(part 1 of 2)
# Autodesk Inventor assembly: Functioning Test Chasis
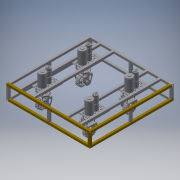
[picture p0: Inventor's stored thumbnail of the model, 180x180]
Saved by Autodesk Inventor 2019 (Build 230136000, 136)
## iProperties
has-driver: False
num-sensors: 0
has-driver: True
driver-type: 1
motor-type: 0
driver-port1: 1
driver-port2: -1
driver-isCan: False
driver-lowerLimit: 0.0
driver-upperLimit: 0.0
driver-inputGear: 0.0
driver-outputGear: 0.0
driver-hasBrake: False
has-wheel: True
wheel-type: 3
wheel-isDriveWheel: True
wheel-frictionLevel: 1
has-pneumatic: False
has-elevator: False
driver-port1: 0
Created: 2019-01-14
Part Number: Functioning Test Chasis
Document SubType Name: Assembly
Designer: josh
robot-name: Chasis
robot-weight-kg: 222.26052856445312
robot-prefer-metric: False
robot-driveTrainType: 1
Author: josh
## Documents named in this file (36)
- D:\Synthesis Robots\Epsilon\Functioning Test Chasis.iam
- D:\Synthesis Robots\Epsilon\Chasis.iam
- D:\Synthesis Robots\Epsilon\4 in HiGrip Wheel.iam
- D:\Synthesis Robots\Epsilon\FR6ZZ-L Hex Bearing.ipt
- D:\Synthesis Robots\Epsilon\375 Hex Output Shaft Rev 2.ipt
- D:\Synthesis Robots\Epsilon\375 Hex Hub.ipt
- D:\Synthesis Robots\Epsilon\10-24 Hex Washer Rolling x 3-4_93882A213.ipt
- D:\Synthesis Robots\Epsilon\125x443 spacer SPS-0750-0443-0125.ipt
- D:\Synthesis Robots\Epsilon\375 E-klip - Mcm 97431A320_97431A320.ipt
- D:\Synthesis Robots\Epsilon\20t 1-25mod bevel gear.ipt
- D:\Synthesis Robots\Epsilon\40t 1-25mod bevel gear.ipt
- D:\Synthesis Robots\Epsilon\AMS C Housing Rev 2.ipt
- D:\Synthesis Robots\Epsilon\10-32 Nylock Nut 1_90631A411.ipt
- D:\Synthesis Robots\Epsilon\10-32x1250_shcs.ipt
- D:\Synthesis Robots\Epsilon\620x215 alum spacer 83062 K-S.ipt
- D:\Synthesis Robots\Epsilon\Bevel Input Shaft.ipt
- D:\Synthesis Robots\Epsilon\FR8ZZ Bearing_smart.ipt
- D:\Synthesis Robots\Epsilon\FR6ZZ Bearing_smart.ipt
- D:\Synthesis Robots\Epsilon\12T CIM Shaft.ipt
- D:\Synthesis Robots\Epsilon\Gear Plate.ipt
- D:\Synthesis Robots\Epsilon\40T 20dp 375h_Inch - Spur gear 20DP 40T 14.5PA .372FW ---S40N3.0H2.0L0.25N.ipt
- D:\Synthesis Robots\Epsilon\500 Washer am-1001.ipt
- D:\Synthesis Robots\Epsilon\10-32x0625_shcs_HX-SHCS 0.19-32x1.375x1-C.ipt
- D:\Synthesis Robots\Epsilon\1100x215 alum spacer 83062 K-S.ipt
- D:\Synthesis Robots\Epsilon\10-32 Nylock Nut.ipt
- D:\Synthesis Robots\Epsilon\10-32x1750_shcs_HX-SHCS 0.19-32x1.375x1-C.ipt
- D:\Synthesis Robots\Epsilon\Bearing Plate.ipt
- D:\Synthesis Robots\Epsilon\40T Sleeve Gear REV2.ipt
- D:\Synthesis Robots\Epsilon\VEX 217-2736 0500 Collar Clamp.ipt
- D:\Synthesis Robots\Epsilon\CIM Motor SW.ipt
- D:\Synthesis Robots\Epsilon\Motor Mount Plate Rev 2.ipt
- D:\Synthesis Robots\Epsilon\48T 10mm bore gear.ipt
- D:\Synthesis Robots\Epsilon\PG-71.ipt
- D:\Synthesis Robots\Epsilon\SHCS M4x10_91290A187.ipt
- D:\Synthesis Robots\Epsilon\438x406 spacer 13RS100043.ipt
- D:\Synthesis Robots\Epsilon\375 External Self Locking Ring_98430A134.ipt
## Components (273 placed, 35 different names)
1. Chasis:1 [sub-assembly] — Mate:253, Flush:23, Mate:254, Mate:505, Flush:46, Mate:506, Mate:507, Flush:47, Mate:508, Mate:634, Flush:59, Mate:635
2. 4 in HiGrip Wheel:2 [sub-assembly]
3. Bevel Input Shaft:2
4. AMS C Housing Rev 2:2
5. FR6ZZ-L Hex Bearing:4
6. 20t 1-25mod bevel gear:2
7. 375 Hex Output Shaft Rev 2:2
8. 375 Hex Hub:2
9. 10-24 Hex Washer Rolling x 3-4_93882A213:7
10. 10-24 Hex Washer Rolling x 3-4_93882A213:8
11. 10-24 Hex Washer Rolling x 3-4_93882A213:9
12. 10-24 Hex Washer Rolling x 3-4_93882A213:10
13. 10-24 Hex Washer Rolling x 3-4_93882A213:11
14. 10-24 Hex Washer Rolling x 3-4_93882A213:12
15. 125x443 spacer SPS-0750-0443-0125:2
16. 375 E-klip - Mcm 97431A320_97431A320:2
17. 40t 1-25mod bevel gear:2
18. FR8ZZ Bearing_smart:2
19. 12T CIM Shaft:2
20. 10-32 Nylock Nut 1_90631A411:5
21. 10-32 Nylock Nut 1_90631A411:6
22. 10-32 Nylock Nut 1_90631A411:7
23. 10-32 Nylock Nut 1_90631A411:8
24. 10-32x1250_shcs:5
25. 10-32x1250_shcs:6
26. 10-32x1250_shcs:7
27. 10-32x1250_shcs:8
28. 620x215 alum spacer 83062 K-S:5
29. 620x215 alum spacer 83062 K-S:6
30. 620x215 alum spacer 83062 K-S:7
31. 620x215 alum spacer 83062 K-S:8
32. FR6ZZ Bearing_smart:3
33. Gear Plate:2
34. 40T 20dp 375h_Inch - Spur gear 20DP 40T 14.5PA .372FW ---S40N3.0H2.0L0.25N:2
35. 500 Washer am-1001:3
36. 500 Washer am-1001:4
37. FR6ZZ Bearing_smart:4
38. 10-32x0625_shcs_HX-SHCS 0.19-32x1.375x1-C:7
39. 10-32x0625_shcs_HX-SHCS 0.19-32x1.375x1-C:8
40. 10-32x0625_shcs_HX-SHCS 0.19-32x1.375x1-C:9
41. 10-32x0625_shcs_HX-SHCS 0.19-32x1.375x1-C:10
42. 40T Sleeve Gear REV2:2
43. PG-71:2
44. 48T 10mm bore gear:2
45. 375 External Self Locking Ring_98430A134:2
46. 438x406 spacer 13RS100043:2
47. SHCS M4x10_91290A187:8
48. SHCS M4x10_91290A187:7
49. SHCS M4x10_91290A187:6
50. SHCS M4x10_91290A187:5
51. 10-32x0625_shcs_HX-SHCS 0.19-32x1.375x1-C:12
52. 10-32x0625_shcs_HX-SHCS 0.19-32x1.375x1-C:11
53. Motor Mount Plate Rev 2:2 — Mate:253, Flush:23, Mate:254
54. CIM Motor SW:2
55. VEX 217-2736 0500 Collar Clamp:2
56. Bearing Plate:2
57. 10-32 Nylock Nut:8
58. 10-32 Nylock Nut:7
59. 10-32 Nylock Nut:6
60. 10-32x1750_shcs_HX-SHCS 0.19-32x1.375x1-C:8
61. 10-32x1750_shcs_HX-SHCS 0.19-32x1.375x1-C:7
62. 10-32x1750_shcs_HX-SHCS 0.19-32x1.375x1-C:6
63. 1100x215 alum spacer 83062 K-S:8
64. 1100x215 alum spacer 83062 K-S:7
65. 1100x215 alum spacer 83062 K-S:6
66. 10-32x1750_shcs_HX-SHCS 0.19-32x1.375x1-C:5
67. 10-32 Nylock Nut:5
68. 1100x215 alum spacer 83062 K-S:5
69. FR6ZZ-L Hex Bearing:3
70. FR6ZZ-L Hex Bearing:5
71. FR6ZZ-L Hex Bearing:6
72. 375 Hex Output Shaft Rev 2:3
73. 375 Hex Hub:3
74. 10-24 Hex Washer Rolling x 3-4_93882A213:13
75. 10-24 Hex Washer Rolling x 3-4_93882A213:14
76. 10-24 Hex Washer Rolling x 3-4_93882A213:15
77. 10-24 Hex Washer Rolling x 3-4_93882A213:16
78. 10-24 Hex Washer Rolling x 3-4_93882A213:17
79. 10-24 Hex Washer Rolling x 3-4_93882A213:18
80. 125x443 spacer SPS-0750-0443-0125:3
81. 375 E-klip - Mcm 97431A320_97431A320:3
82. 20t 1-25mod bevel gear:3
83. 40t 1-25mod bevel gear:3
84. AMS C Housing Rev 2:3
85. 10-32 Nylock Nut 1_90631A411:9
86. 10-32 Nylock Nut 1_90631A411:10
87. 10-32 Nylock Nut 1_90631A411:11
88. 10-32 Nylock Nut 1_90631A411:12
89. 10-32x1250_shcs:9
90. 10-32x1250_shcs:10
91. 10-32x1250_shcs:11
92. 10-32x1250_shcs:12
93. 620x215 alum spacer 83062 K-S:9
94. 620x215 alum spacer 83062 K-S:10
95. 620x215 alum spacer 83062 K-S:11
96. 620x215 alum spacer 83062 K-S:12
97. Bevel Input Shaft:3
98. FR8ZZ Bearing_smart:3
99. FR6ZZ Bearing_smart:5
100. 12T CIM Shaft:3
101. Gear Plate:3
102. 40T 20dp 375h_Inch - Spur gear 20DP 40T 14.5PA .372FW ---S40N3.0H2.0L0.25N:3
103. 500 Washer am-1001:5
104. 500 Washer am-1001:6
105. FR6ZZ Bearing_smart:6
106. 10-32x0625_shcs_HX-SHCS 0.19-32x1.375x1-C:13
107. 10-32x0625_shcs_HX-SHCS 0.19-32x1.375x1-C:14
108. 10-32x0625_shcs_HX-SHCS 0.19-32x1.375x1-C:15
109. 10-32x0625_shcs_HX-SHCS 0.19-32x1.375x1-C:16
110. 1100x215 alum spacer 83062 K-S:9
111. 10-32 Nylock Nut:9
112. 10-32x1750_shcs_HX-SHCS 0.19-32x1.375x1-C:9
113. 1100x215 alum spacer 83062 K-S:10
114. 1100x215 alum spacer 83062 K-S:11
115. 1100x215 alum spacer 83062 K-S:12
116. 10-32x1750_shcs_HX-SHCS 0.19-32x1.375x1-C:10
117. 10-32x1750_shcs_HX-SHCS 0.19-32x1.375x1-C:11
118. 10-32x1750_shcs_HX-SHCS 0.19-32x1.375x1-C:12
119. 10-32 Nylock Nut:10
120. 10-32 Nylock Nut:11
121. 10-32 Nylock Nut:12
122. Bearing Plate:3
123. 40T Sleeve Gear REV2:3
124. VEX 217-2736 0500 Collar Clamp:3
125. CIM Motor SW:3
126. Motor Mount Plate Rev 2:3 — Mate:505, Flush:46, Mate:506
127. 48T 10mm bore gear:3
128. 10-32x0625_shcs_HX-SHCS 0.19-32x1.375x1-C:17
129. 10-32x0625_shcs_HX-SHCS 0.19-32x1.375x1-C:18
130. PG-71:3
131. SHCS M4x10_91290A187:9
132. SHCS M4x10_91290A187:10
133. SHCS M4x10_91290A187:11
134. SHCS M4x10_91290A187:12
135. 438x406 spacer 13RS100043:3
136. 375 External Self Locking Ring_98430A134:3
137. 4 in HiGrip Wheel:3 [sub-assembly]
138. FR6ZZ-L Hex Bearing:7
139. FR6ZZ-L Hex Bearing:8
140. 375 Hex Output Shaft Rev 2:4
141. 375 Hex Hub:4
142. 10-24 Hex Washer Rolling x 3-4_93882A213:19
143. 10-24 Hex Washer Rolling x 3-4_93882A213:20
144. 10-24 Hex Washer Rolling x 3-4_93882A213:21
145. 10-24 Hex Washer Rolling x 3-4_93882A213:22
146. 10-24 Hex Washer Rolling x 3-4_93882A213:23
147. 10-24 Hex Washer Rolling x 3-4_93882A213:24
148. 125x443 spacer SPS-0750-0443-0125:4
149. 375 E-klip - Mcm 97431A320_97431A320:4
150. 20t 1-25mod bevel gear:4
151. 40t 1-25mod bevel gear:4
152. AMS C Housing Rev 2:4
153. 10-32 Nylock Nut 1_90631A411:13
154. 10-32 Nylock Nut 1_90631A411:14
155. 10-32 Nylock Nut 1_90631A411:15
156. 10-32 Nylock Nut 1_90631A411:16
157. 10-32x1250_shcs:13
158. 10-32x1250_shcs:14
159. 10-32x1250_shcs:15
160. 10-32x1250_shcs:16
161. 620x215 alum spacer 83062 K-S:13
162. 620x215 alum spacer 83062 K-S:14
163. 620x215 alum spacer 83062 K-S:15
164. 620x215 alum spacer 83062 K-S:16
165. Bevel Input Shaft:4
166. FR8ZZ Bearing_smart:4
167. FR6ZZ Bearing_smart:7
168. 12T CIM Shaft:4
169. Gear Plate:4
170. 40T 20dp 375h_Inch - Spur gear 20DP 40T 14.5PA .372FW ---S40N3.0H2.0L0.25N:4
171. 500 Washer am-1001:7
172. 500 Washer am-1001:8
173. FR6ZZ Bearing_smart:8
174. 10-32x0625_shcs_HX-SHCS 0.19-32x1.375x1-C:19
175. 10-32x0625_shcs_HX-SHCS 0.19-32x1.375x1-C:20
176. 10-32x0625_shcs_HX-SHCS 0.19-32x1.375x1-C:21
177. 10-32x0625_shcs_HX-SHCS 0.19-32x1.375x1-C:22
178. 1100x215 alum spacer 83062 K-S:13
179. 10-32 Nylock Nut:13
180. 10-32x1750_shcs_HX-SHCS 0.19-32x1.375x1-C:13
181. 1100x215 alum spacer 83062 K-S:14
182. 1100x215 alum spacer 83062 K-S:15
183. 1100x215 alum spacer 83062 K-S:16
184. 10-32x1750_shcs_HX-SHCS 0.19-32x1.375x1-C:14
185. 10-32x1750_shcs_HX-SHCS 0.19-32x1.375x1-C:15
186. 10-32x1750_shcs_HX-SHCS 0.19-32x1.375x1-C:16
187. 10-32 Nylock Nut:14
188. 10-32 Nylock Nut:15
189. 10-32 Nylock Nut:16
190. Bearing Plate:4
191. 40T Sleeve Gear REV2:4
192. VEX 217-2736 0500 Collar Clamp:4
193. CIM Motor SW:4
194. Motor Mount Plate Rev 2:4 — Mate:507, Flush:47, Mate:508
195. 48T 10mm bore gear:4
196. 10-32x0625_shcs_HX-SHCS 0.19-32x1.375x1-C:23
197. 10-32x0625_shcs_HX-SHCS 0.19-32x1.375x1-C:24
198. PG-71:4
199. SHCS M4x10_91290A187:13
200. SHCS M4x10_91290A187:14
201. SHCS M4x10_91290A187:15
202. SHCS M4x10_91290A187:16
203. 438x406 spacer 13RS100043:4
204. 375 External Self Locking Ring_98430A134:4
205. 4 in HiGrip Wheel:4 [sub-assembly]
206. FR6ZZ-L Hex Bearing:9
207. FR6ZZ-L Hex Bearing:10
208. 375 Hex Output Shaft Rev 2:5
209. 375 Hex Hub:5
210. 10-24 Hex Washer Rolling x 3-4_93882A213:25
211. 10-24 Hex Washer Rolling x 3-4_93882A213:26
212. 10-24 Hex Washer Rolling x 3-4_93882A213:27
213. 10-24 Hex Washer Rolling x 3-4_93882A213:28
214. 10-24 Hex Washer Rolling x 3-4_93882A213:29
215. 10-24 Hex Washer Rolling x 3-4_93882A213:30
216. 125x443 spacer SPS-0750-0443-0125:5
217. 375 E-klip - Mcm 97431A320_97431A320:5
218. 20t 1-25mod bevel gear:5
219. 40t 1-25mod bevel gear:5
220. AMS C Housing Rev 2:5
221. 10-32 Nylock Nut 1_90631A411:17
222. 10-32 Nylock Nut 1_90631A411:18
223. 10-32 Nylock Nut 1_90631A411:19
224. 10-32 Nylock Nut 1_90631A411:20
225. 10-32x1250_shcs:17
226. 10-32x1250_shcs:18
227. 10-32x1250_shcs:19
228. 10-32x1250_shcs:20
229. 620x215 alum spacer 83062 K-S:17
230. 620x215 alum spacer 83062 K-S:18
231. 620x215 alum spacer 83062 K-S:19
232. 620x215 alum spacer 83062 K-S:20
233. Bevel Input Shaft:5
234. FR8ZZ Bearing_smart:5
235. FR6ZZ Bearing_smart:9
236. 12T CIM Shaft:5
237. Gear Plate:5
238. 40T 20dp 375h_Inch - Spur gear 20DP 40T 14.5PA .372FW ---S40N3.0H2.0L0.25N:5
239. 500 Washer am-1001:9
240. 500 Washer am-1001:10
241. FR6ZZ Bearing_smart:10
242. 10-32x0625_shcs_HX-SHCS 0.19-32x1.375x1-C:25
243. 10-32x0625_shcs_HX-SHCS 0.19-32x1.375x1-C:26
244. 10-32x0625_shcs_HX-SHCS 0.19-32x1.375x1-C:27
245. 10-32x0625_shcs_HX-SHCS 0.19-32x1.375x1-C:28
246. 1100x215 alum spacer 83062 K-S:17
247. 10-32 Nylock Nut:17
248. 10-32x1750_shcs_HX-SHCS 0.19-32x1.375x1-C:17
249. 1100x215 alum spacer 83062 K-S:18
250. 1100x215 alum spacer 83062 K-S:19
251. 1100x215 alum spacer 83062 K-S:20
252. 10-32x1750_shcs_HX-SHCS 0.19-32x1.375x1-C:18
253. 10-32x1750_shcs_HX-SHCS 0.19-32x1.375x1-C:19
254. 10-32x1750_shcs_HX-SHCS 0.19-32x1.375x1-C:20
255. 10-32 Nylock Nut:18
256. 10-32 Nylock Nut:19
257. 10-32 Nylock Nut:20
258. Bearing Plate:5
259. 40T Sleeve Gear REV2:5
260. VEX 217-2736 0500 Collar Clamp:5
261. CIM Motor SW:5
262. Motor Mount Plate Rev 2:5 — Mate:634, Flush:59, Mate:635
263. 48T 10mm bore gear:5
264. 10-32x0625_shcs_HX-SHCS 0.19-32x1.375x1-C:29
265. 10-32x0625_shcs_HX-SHCS 0.19-32x1.375x1-C:30
266. PG-71:5
267. SHCS M4x10_91290A187:17
268. SHCS M4x10_91290A187:18
269. SHCS M4x10_91290A187:19
270. SHCS M4x10_91290A187:20
271. 438x406 spacer 13RS100043:5
272. 375 External Self Locking Ring_98430A134:5
273. 4 in HiGrip Wheel:5 [sub-assembly]
## Relationships (592: Mate 508, Flush 48, RevoluteJoint 28, RelateRotation 8)
- [Mate]: 375 Hex Hub:2 ↔ 10-24 Hex Washer Rolling x 3-4_93882A213:12
- [Mate]: 375 Hex Hub:2 ↔ 10-24 Hex Washer Rolling x 3-4_93882A213:7
- [Mate]: 375 Hex Hub:2 ↔ 10-24 Hex Washer Rolling x 3-4_93882A213:11
- [Mate]: 375 Hex Hub:2 ↔ 10-24 Hex Washer Rolling x 3-4_93882A213:10
- [Mate]: 375 Hex Hub:2 ↔ 10-24 Hex Washer Rolling x 3-4_93882A213:9
- [Mate]: 375 Hex Hub:2 ↔ 10-24 Hex Washer Rolling x 3-4_93882A213:8
- [Mate]: 375 Hex Hub:2 ↔ 10-24 Hex Washer Rolling x 3-4_93882A213:8
- [Mate]: 375 Hex Hub:2 ↔ 10-24 Hex Washer Rolling x 3-4_93882A213:10
- [Mate]: 375 Hex Hub:2 ↔ 10-24 Hex Washer Rolling x 3-4_93882A213:9
- [Mate]: 375 Hex Hub:2 ↔ 10-24 Hex Washer Rolling x 3-4_93882A213:7
- [Mate]: 375 Hex Hub:2 ↔ 10-24 Hex Washer Rolling x 3-4_93882A213:12
- [Mate]: 375 Hex Hub:2 ↔ 10-24 Hex Washer Rolling x 3-4_93882A213:11
- [Mate]: 375 Hex Output Shaft Rev 2:2 ↔ 375 Hex Hub:2
- [Mate]: 375 Hex Output Shaft Rev 2:2 ↔ 375 Hex Hub:2
- [Mate]: 375 Hex Output Shaft Rev 2:2 ↔ FR6ZZ-L Hex Bearing:3
- [Mate]: 375 Hex Output Shaft Rev 2:2 ↔ FR6ZZ-L Hex Bearing:3
- [Mate]: 375 Hex Output Shaft Rev 2:2 ↔ 40t 1-25mod bevel gear:2
- [Mate]: 375 Hex Output Shaft Rev 2:2 ↔ 40t 1-25mod bevel gear:2
- [RevoluteJoint]: AMS C Housing Rev 2:2 ↔ FR6ZZ-L Hex Bearing:4
- [RevoluteJoint]: AMS C Housing Rev 2:2 ↔ FR6ZZ-L Hex Bearing:3
- [Mate]: 125x443 spacer SPS-0750-0443-0125:2 ↔ FR6ZZ-L Hex Bearing:3
- [Mate]: 125x443 spacer SPS-0750-0443-0125:2 ↔ FR6ZZ-L Hex Bearing:3
- [Mate]: 375 Hex Output Shaft Rev 2:2 ↔ 375 E-klip - Mcm 97431A320_97431A320:2
- [Mate]: 375 Hex Output Shaft Rev 2:2 ↔ 375 E-klip - Mcm 97431A320_97431A320:2
- [Mate]: 375 Hex Hub:2 ↔ 125x443 spacer SPS-0750-0443-0125:2
- [Flush]: 375 Hex Output Shaft Rev 2:2 ↔ FR6ZZ-L Hex Bearing:3
- [RevoluteJoint]: 10-32 Nylock Nut 1_90631A411:5 ↔ 10-32x1250_shcs:7
- [RevoluteJoint]: 10-32 Nylock Nut 1_90631A411:6 ↔ 10-32x1250_shcs:8
- [RevoluteJoint]: 10-32 Nylock Nut 1_90631A411:8 ↔ 10-32x1250_shcs:6
- [RevoluteJoint]: 10-32 Nylock Nut 1_90631A411:7 ↔ 10-32x1250_shcs:5
- [Mate]: 10-32x1250_shcs:6 ↔ Gear Plate:2
- [Mate]: 10-32x1250_shcs:6 ↔ 620x215 alum spacer 83062 K-S:6
- [Flush]: 10-32x1250_shcs:6 ↔ Gear Plate:2
- [Mate]: 620x215 alum spacer 83062 K-S:6 ↔ Gear Plate:2
- [Mate]: 10-32x1250_shcs:5 ↔ Gear Plate:2
- [Mate]: 10-32x1250_shcs:5 ↔ 620x215 alum spacer 83062 K-S:5
- [Flush]: 10-32x1250_shcs:5 ↔ Gear Plate:2
- [Mate]: 620x215 alum spacer 83062 K-S:5 ↔ Gear Plate:2
- [Mate]: 10-32x1250_shcs:7 ↔ Gear Plate:2
- [Flush]: 10-32x1250_shcs:7 ↔ Gear Plate:2
- [Mate]: 10-32x1250_shcs:7 ↔ 620x215 alum spacer 83062 K-S:7
- [Mate]: 620x215 alum spacer 83062 K-S:7 ↔ Gear Plate:2
- [Mate]: 10-32x1250_shcs:8 ↔ 620x215 alum spacer 83062 K-S:8
- [Flush]: 10-32x1250_shcs:8 ↔ Gear Plate:2
- [Mate]: 10-32x1250_shcs:8 ↔ Gear Plate:2
- [Mate]: 620x215 alum spacer 83062 K-S:8 ↔ Gear Plate:2
- [Mate]: FR8ZZ Bearing_smart:2 ↔ 12T CIM Shaft:2
- [Mate]: FR8ZZ Bearing_smart:2 ↔ 12T CIM Shaft:2
- [Mate]: 12T CIM Shaft:2 ↔ Gear Plate:2
- [Mate]: Bevel Input Shaft:2 ↔ FR6ZZ Bearing_smart:3
- [Mate]: Bevel Input Shaft:2 ↔ 500 Washer am-1001:3
- [Mate]: Bevel Input Shaft:2 ↔ 40T 20dp 375h_Inch - Spur gear 20DP 40T 14.5PA .372FW ---S40N3.0H2.0L0.25N:2
- [Mate]: Bevel Input Shaft:2 ↔ 40T 20dp 375h_Inch - Spur gear 20DP 40T 14.5PA .372FW ---S40N3.0H2.0L0.25N:2
- [Flush]: Bevel Input Shaft:2 ↔ 40T 20dp 375h_Inch - Spur gear 20DP 40T 14.5PA .372FW ---S40N3.0H2.0L0.25N:2
- [Mate]: Bevel Input Shaft:2 ↔ 500 Washer am-1001:4
- [Mate]: Bevel Input Shaft:2 ↔ FR6ZZ Bearing_smart:4
- [Mate]: 500 Washer am-1001:4 ↔ FR6ZZ Bearing_smart:4
- [Mate]: Bevel Input Shaft:2 ↔ 500 Washer am-1001:4
- [Flush]: Bevel Input Shaft:2 ↔ 500 Washer am-1001:3
- [Mate]: Gear Plate:2 ↔ FR6ZZ Bearing_smart:4
- [Mate]: Gear Plate:2 ↔ FR6ZZ Bearing_smart:4
- [RevoluteJoint]: Bevel Input Shaft:2 ↔ 20t 1-25mod bevel gear:2
- [Mate]: Gear Plate:2 ↔ 10-32x0625_shcs_HX-SHCS 0.19-32x1.375x1-C:9
- [Flush]: Gear Plate:2 ↔ 10-32x0625_shcs_HX-SHCS 0.19-32x1.375x1-C:9
- [Mate]: Gear Plate:2 ↔ 10-32x0625_shcs_HX-SHCS 0.19-32x1.375x1-C:8
- [Flush]: Gear Plate:2 ↔ 10-32x0625_shcs_HX-SHCS 0.19-32x1.375x1-C:8
- [Mate]: Gear Plate:2 ↔ 10-32x0625_shcs_HX-SHCS 0.19-32x1.375x1-C:7
- [Flush]: Gear Plate:2 ↔ 10-32x0625_shcs_HX-SHCS 0.19-32x1.375x1-C:7
- [Mate]: Gear Plate:2 ↔ 10-32x0625_shcs_HX-SHCS 0.19-32x1.375x1-C:10
- [Flush]: Gear Plate:2 ↔ 10-32x0625_shcs_HX-SHCS 0.19-32x1.375x1-C:10
- [Mate]: FR6ZZ Bearing_smart:3 ↔ 500 Washer am-1001:3
- [Mate]: AMS C Housing Rev 2:2 ↔ 10-32x1250_shcs:6
- [Mate]: AMS C Housing Rev 2:2 ↔ 10-32x1250_shcs:5
- [Mate]: AMS C Housing Rev 2:2 ↔ FR6ZZ Bearing_smart:3
- [Mate]: AMS C Housing Rev 2:2 ↔ FR8ZZ Bearing_smart:2
- [Mate]: 10-32x0625_shcs_HX-SHCS 0.19-32x1.375x1-C:9 ↔ 40T Sleeve Gear REV2:2
- [Mate]: 10-32x0625_shcs_HX-SHCS 0.19-32x1.375x1-C:10 ↔ 40T Sleeve Gear REV2:2
- [Mate]: 10-32x0625_shcs_HX-SHCS 0.19-32x1.375x1-C:7 ↔ 40T Sleeve Gear REV2:2
- [Mate]: 10-32x0625_shcs_HX-SHCS 0.19-32x1.375x1-C:8 ↔ 40T Sleeve Gear REV2:2
- [Mate]: 12T CIM Shaft:2 ↔ 40T Sleeve Gear REV2:2
- [Mate]: Gear Plate:2 ↔ 40T Sleeve Gear REV2:2
- [Mate]: 10-32x1750_shcs_HX-SHCS 0.19-32x1.375x1-C:5 ↔ 10-32 Nylock Nut:5
- [Mate]: 10-32 Nylock Nut:6 ↔ 10-32x1750_shcs_HX-SHCS 0.19-32x1.375x1-C:8
- [Mate]: 10-32 Nylock Nut:8 ↔ 10-32x1750_shcs_HX-SHCS 0.19-32x1.375x1-C:7
- [Mate]: 10-32 Nylock Nut:7 ↔ 10-32x1750_shcs_HX-SHCS 0.19-32x1.375x1-C:6
- [Mate]: 10-32x1750_shcs_HX-SHCS 0.19-32x1.375x1-C:7 ↔ 1100x215 alum spacer 83062 K-S:7
- [Mate]: Bearing Plate:2 ↔ 10-32x1750_shcs_HX-SHCS 0.19-32x1.375x1-C:7
- [Mate]: Bearing Plate:2 ↔ 10-32x1750_shcs_HX-SHCS 0.19-32x1.375x1-C:7
- [Mate]: 10-32x1750_shcs_HX-SHCS 0.19-32x1.375x1-C:8 ↔ 1100x215 alum spacer 83062 K-S:6
- [Mate]: Bearing Plate:2 ↔ 10-32x1750_shcs_HX-SHCS 0.19-32x1.375x1-C:8
- [Mate]: Bearing Plate:2 ↔ 1100x215 alum spacer 83062 K-S:6
- [Mate]: Bearing Plate:2 ↔ 10-32x1750_shcs_HX-SHCS 0.19-32x1.375x1-C:8
- [Mate]: Motor Mount Plate Rev 2:2 ↔ 10-32 Nylock Nut:6
- [Mate]: Bearing Plate:2 ↔ 1100x215 alum spacer 83062 K-S:7
- [Mate]: Motor Mount Plate Rev 2:2 ↔ 10-32 Nylock Nut:8
- [Mate]: Bearing Plate:2 ↔ 10-32x1750_shcs_HX-SHCS 0.19-32x1.375x1-C:5
- [Mate]: 10-32x1750_shcs_HX-SHCS 0.19-32x1.375x1-C:5 ↔ 10-32 Nylock Nut:5
- [Mate]: Motor Mount Plate Rev 2:2 ↔ 10-32 Nylock Nut:5
- [Mate]: Bearing Plate:2 ↔ 10-32x1750_shcs_HX-SHCS 0.19-32x1.375x1-C:5
- [Mate]: 10-32x1750_shcs_HX-SHCS 0.19-32x1.375x1-C:5 ↔ 1100x215 alum spacer 83062 K-S:5
- [Mate]: Bearing Plate:2 ↔ 1100x215 alum spacer 83062 K-S:5
- [Mate]: Bearing Plate:2 ↔ 10-32x1750_shcs_HX-SHCS 0.19-32x1.375x1-C:6
- [Mate]: Bearing Plate:2 ↔ 10-32x1750_shcs_HX-SHCS 0.19-32x1.375x1-C:6
- [Mate]: 10-32x1750_shcs_HX-SHCS 0.19-32x1.375x1-C:6 ↔ 1100x215 alum spacer 83062 K-S:8
- [Mate]: Bearing Plate:2 ↔ 1100x215 alum spacer 83062 K-S:8
- [Mate]: Motor Mount Plate Rev 2:2 ↔ 10-32 Nylock Nut:7
- [Mate]: 10-32x0625_shcs_HX-SHCS 0.19-32x1.375x1-C:12 ↔ CIM Motor SW:2
- [Mate]: 10-32x0625_shcs_HX-SHCS 0.19-32x1.375x1-C:12 ↔ Motor Mount Plate Rev 2:2
- [Mate]: 10-32x0625_shcs_HX-SHCS 0.19-32x1.375x1-C:12 ↔ Motor Mount Plate Rev 2:2
- [Mate]: 10-32x0625_shcs_HX-SHCS 0.19-32x1.375x1-C:11 ↔ CIM Motor SW:2
- [Mate]: 10-32x0625_shcs_HX-SHCS 0.19-32x1.375x1-C:11 ↔ Motor Mount Plate Rev 2:2
- [Mate]: 10-32x0625_shcs_HX-SHCS 0.19-32x1.375x1-C:11 ↔ Motor Mount Plate Rev 2:2
- [Mate]: 12T CIM Shaft:2 ↔ CIM Motor SW:2
- [Mate]: CIM Motor SW:2 ↔ VEX 217-2736 0500 Collar Clamp:2
- [Mate]: Motor Mount Plate Rev 2:2 ↔ VEX 217-2736 0500 Collar Clamp:2
- [Mate]: 12T CIM Shaft:2 ↔ CIM Motor SW:2
- [Mate]: Motor Mount Plate Rev 2:2 ↔ CIM Motor SW:2
- [Mate]: PG-71:2 ↔ 375 External Self Locking Ring_98430A134:2
- [Mate]: PG-71:2 ↔ 48T 10mm bore gear:2
- [Mate]: Motor Mount Plate Rev 2:2 ↔ 10-32x1750_shcs_HX-SHCS 0.19-32x1.375x1-C:5
- [Mate]: Motor Mount Plate Rev 2:2 ↔ 10-32x1750_shcs_HX-SHCS 0.19-32x1.375x1-C:8
- [Mate]: Motor Mount Plate Rev 2:2 ↔ 1100x215 alum spacer 83062 K-S:5
- [Mate]: PG-71:2 ↔ 438x406 spacer 13RS100043:2
- [Mate]: 438x406 spacer 13RS100043:2 ↔ Motor Mount Plate Rev 2:2
- [Mate]: SHCS M4x10_91290A187:6 ↔ Motor Mount Plate Rev 2:2
- [Mate]: SHCS M4x10_91290A187:5 ↔ Motor Mount Plate Rev 2:2
- [Mate]: SHCS M4x10_91290A187:8 ↔ Motor Mount Plate Rev 2:2
- [Mate]: SHCS M4x10_91290A187:7 ↔ Motor Mount Plate Rev 2:2
- [Mate]: SHCS M4x10_91290A187:5 ↔ Motor Mount Plate Rev 2:2
- [Mate]: SHCS M4x10_91290A187:6 ↔ Motor Mount Plate Rev 2:2
- [Mate]: SHCS M4x10_91290A187:8 ↔ Motor Mount Plate Rev 2:2
- [Mate]: SHCS M4x10_91290A187:7 ↔ Motor Mount Plate Rev 2:2
- [Mate]: PG-71:2 ↔ 438x406 spacer 13RS100043:2
- [Mate]: PG-71:2 ↔ Motor Mount Plate Rev 2:2
- [Mate]: 48T 10mm bore gear:2 ↔ 438x406 spacer 13RS100043:2
- [Mate]: PG-71:2 ↔ 375 External Self Locking Ring_98430A134:2
- [RelateRotation] (1 ul): 20t 1-25mod bevel gear:2 ↔ 40t 1-25mod bevel gear:2
- [Mate]: Bevel Input Shaft:2 ↔ 20t 1-25mod bevel gear:2
- [RelateRotation] (1 ul): 40T Sleeve Gear REV2:2 ↔ 48T 10mm bore gear:2
- [Mate]: PG-71:2 ↔ 48T 10mm bore gear:2
- [Mate]: 4 in HiGrip Wheel:2 ↔ 10-24 Hex Washer Rolling x 3-4_93882A213:12
- [Mate]: 4 in HiGrip Wheel:2 ↔ 10-24 Hex Washer Rolling x 3-4_93882A213:11
- [Mate]: 4 in HiGrip Wheel:2 ↔ 10-24 Hex Washer Rolling x 3-4_93882A213:10
- [Mate]: 4 in HiGrip Wheel:2 ↔ 375 Hex Hub:2
- [Mate]: 4 in HiGrip Wheel:2 ↔ 40t 1-25mod bevel gear:2
- Mate:253: Chasis:1 ↔ Motor Mount Plate Rev 2:2
- Flush:23: Chasis:1 ↔ Motor Mount Plate Rev 2:2
- Mate:254 (95.25 mm): Chasis:1 ↔ Motor Mount Plate Rev 2:2
- [Mate]: 375 Hex Hub:3 ↔ 10-24 Hex Washer Rolling x 3-4_93882A213:18
- [Mate]: 375 Hex Hub:3 ↔ 10-24 Hex Washer Rolling x 3-4_93882A213:13
- [Mate]: 375 Hex Hub:3 ↔ 10-24 Hex Washer Rolling x 3-4_93882A213:17
- [Mate]: 375 Hex Hub:3 ↔ 10-24 Hex Washer Rolling x 3-4_93882A213:16
- [Mate]: 375 Hex Hub:3 ↔ 10-24 Hex Washer Rolling x 3-4_93882A213:15
- [Mate]: 375 Hex Hub:3 ↔ 10-24 Hex Washer Rolling x 3-4_93882A213:14
- [Mate]: 375 Hex Hub:3 ↔ 10-24 Hex Washer Rolling x 3-4_93882A213:14
- [Mate]: 375 Hex Hub:3 ↔ 10-24 Hex Washer Rolling x 3-4_93882A213:16
- [Mate]: 375 Hex Hub:3 ↔ 10-24 Hex Washer Rolling x 3-4_93882A213:15
- [Mate]: 375 Hex Hub:3 ↔ 10-24 Hex Washer Rolling x 3-4_93882A213:13
- [Mate]: 375 Hex Hub:3 ↔ 10-24 Hex Washer Rolling x 3-4_93882A213:18
- [Mate]: 375 Hex Hub:3 ↔ 10-24 Hex Washer Rolling x 3-4_93882A213:17
- [Mate]: 375 Hex Output Shaft Rev 2:3 ↔ 375 Hex Hub:3
- [Mate]: 375 Hex Output Shaft Rev 2:3 ↔ 375 Hex Hub:3
- [Mate]: FR6ZZ-L Hex Bearing:5 ↔ 375 Hex Output Shaft Rev 2:3
- [Mate]: FR6ZZ-L Hex Bearing:5 ↔ 375 Hex Output Shaft Rev 2:3
- [Mate]: 375 Hex Output Shaft Rev 2:3 ↔ 40t 1-25mod bevel gear:3
- [Mate]: 375 Hex Output Shaft Rev 2:3 ↔ 40t 1-25mod bevel gear:3
- [RevoluteJoint]: FR6ZZ-L Hex Bearing:6 ↔ AMS C Housing Rev 2:3
- [RevoluteJoint]: FR6ZZ-L Hex Bearing:5 ↔ AMS C Housing Rev 2:3
- [Mate]: FR6ZZ-L Hex Bearing:5 ↔ 125x443 spacer SPS-0750-0443-0125:3
- [Mate]: FR6ZZ-L Hex Bearing:5 ↔ 125x443 spacer SPS-0750-0443-0125:3
- [Mate]: 375 Hex Output Shaft Rev 2:3 ↔ 375 E-klip - Mcm 97431A320_97431A320:3
- [Mate]: 375 Hex Output Shaft Rev 2:3 ↔ 375 E-klip - Mcm 97431A320_97431A320:3
- [Mate]: 375 Hex Hub:3 ↔ 125x443 spacer SPS-0750-0443-0125:3
- [Flush]: FR6ZZ-L Hex Bearing:5 ↔ 375 Hex Output Shaft Rev 2:3
- [RevoluteJoint]: 10-32 Nylock Nut 1_90631A411:9 ↔ 10-32x1250_shcs:11
- [RevoluteJoint]: 10-32 Nylock Nut 1_90631A411:10 ↔ 10-32x1250_shcs:12
- [RevoluteJoint]: 10-32 Nylock Nut 1_90631A411:12 ↔ 10-32x1250_shcs:10
- [RevoluteJoint]: 10-32 Nylock Nut 1_90631A411:11 ↔ 10-32x1250_shcs:9
- [Mate]: 10-32x1250_shcs:10 ↔ Gear Plate:3
- [Mate]: 10-32x1250_shcs:10 ↔ 620x215 alum spacer 83062 K-S:10
- [Flush]: 10-32x1250_shcs:10 ↔ Gear Plate:3
- [Mate]: 620x215 alum spacer 83062 K-S:10 ↔ Gear Plate:3
- [Mate]: 10-32x1250_shcs:9 ↔ Gear Plate:3
- [Mate]: 10-32x1250_shcs:9 ↔ 620x215 alum spacer 83062 K-S:9
- [Flush]: 10-32x1250_shcs:9 ↔ Gear Plate:3
- [Mate]: 620x215 alum spacer 83062 K-S:9 ↔ Gear Plate:3
- [Mate]: 10-32x1250_shcs:11 ↔ Gear Plate:3
- [Flush]: 10-32x1250_shcs:11 ↔ Gear Plate:3
- [Mate]: 10-32x1250_shcs:11 ↔ 620x215 alum spacer 83062 K-S:11
- [Mate]: 620x215 alum spacer 83062 K-S:11 ↔ Gear Plate:3
- [Mate]: 10-32x1250_shcs:12 ↔ 620x215 alum spacer 83062 K-S:12
- [Flush]: 10-32x1250_shcs:12 ↔ Gear Plate:3
- [Mate]: 10-32x1250_shcs:12 ↔ Gear Plate:3
- [Mate]: 620x215 alum spacer 83062 K-S:12 ↔ Gear Plate:3
- [Mate]: FR8ZZ Bearing_smart:3 ↔ 12T CIM Shaft:3
- [Mate]: FR8ZZ Bearing_smart:3 ↔ 12T CIM Shaft:3
- [Mate]: 12T CIM Shaft:3 ↔ Gear Plate:3
- [Mate]: Bevel Input Shaft:3 ↔ FR6ZZ Bearing_smart:5
- [Mate]: Bevel Input Shaft:3 ↔ 500 Washer am-1001:5
- [Mate]: Bevel Input Shaft:3 ↔ 40T 20dp 375h_Inch - Spur gear 20DP 40T 14.5PA .372FW ---S40N3.0H2.0L0.25N:3
- [Mate]: Bevel Input Shaft:3 ↔ 40T 20dp 375h_Inch - Spur gear 20DP 40T 14.5PA .372FW ---S40N3.0H2.0L0.25N:3
- [Flush]: Bevel Input Shaft:3 ↔ 40T 20dp 375h_Inch - Spur gear 20DP 40T 14.5PA .372FW ---S40N3.0H2.0L0.25N:3
- [Mate]: Bevel Input Shaft:3 ↔ 500 Washer am-1001:6
- [Mate]: Bevel Input Shaft:3 ↔ FR6ZZ Bearing_smart:6
- [Mate]: 500 Washer am-1001:6 ↔ FR6ZZ Bearing_smart:6
- [Mate]: Bevel Input Shaft:3 ↔ 500 Washer am-1001:6
- [Flush]: Bevel Input Shaft:3 ↔ 500 Washer am-1001:5
- [Mate]: Gear Plate:3 ↔ FR6ZZ Bearing_smart:6
- [Mate]: Gear Plate:3 ↔ FR6ZZ Bearing_smart:6
- [RevoluteJoint]: 20t 1-25mod bevel gear:3 ↔ Bevel Input Shaft:3
- [Mate]: Gear Plate:3 ↔ 10-32x0625_shcs_HX-SHCS 0.19-32x1.375x1-C:15
- [Flush]: Gear Plate:3 ↔ 10-32x0625_shcs_HX-SHCS 0.19-32x1.375x1-C:15
- [Mate]: Gear Plate:3 ↔ 10-32x0625_shcs_HX-SHCS 0.19-32x1.375x1-C:14
- [Flush]: Gear Plate:3 ↔ 10-32x0625_shcs_HX-SHCS 0.19-32x1.375x1-C:14
- [Mate]: Gear Plate:3 ↔ 10-32x0625_shcs_HX-SHCS 0.19-32x1.375x1-C:13
- [Flush]: Gear Plate:3 ↔ 10-32x0625_shcs_HX-SHCS 0.19-32x1.375x1-C:13
- [Mate]: Gear Plate:3 ↔ 10-32x0625_shcs_HX-SHCS 0.19-32x1.375x1-C:16
- [Flush]: Gear Plate:3 ↔ 10-32x0625_shcs_HX-SHCS 0.19-32x1.375x1-C:16
- [Mate]: FR6ZZ Bearing_smart:5 ↔ 500 Washer am-1001:5
- [Mate]: AMS C Housing Rev 2:3 ↔ 10-32x1250_shcs:10
- [Mate]: AMS C Housing Rev 2:3 ↔ 10-32x1250_shcs:9
- [Mate]: AMS C Housing Rev 2:3 ↔ FR6ZZ Bearing_smart:5
- [Mate]: AMS C Housing Rev 2:3 ↔ FR8ZZ Bearing_smart:3
- [Mate]: 10-32x0625_shcs_HX-SHCS 0.19-32x1.375x1-C:15 ↔ 40T Sleeve Gear REV2:3
- [Mate]: 10-32x0625_shcs_HX-SHCS 0.19-32x1.375x1-C:16 ↔ 40T Sleeve Gear REV2:3
- [Mate]: 10-32x0625_shcs_HX-SHCS 0.19-32x1.375x1-C:13 ↔ 40T Sleeve Gear REV2:3
- [Mate]: 10-32x0625_shcs_HX-SHCS 0.19-32x1.375x1-C:14 ↔ 40T Sleeve Gear REV2:3
- [Mate]: 12T CIM Shaft:3 ↔ 40T Sleeve Gear REV2:3
- [Mate]: Gear Plate:3 ↔ 40T Sleeve Gear REV2:3
- [Mate]: 10-32 Nylock Nut:9 ↔ 10-32x1750_shcs_HX-SHCS 0.19-32x1.375x1-C:9
- [Mate]: 10-32x1750_shcs_HX-SHCS 0.19-32x1.375x1-C:12 ↔ 10-32 Nylock Nut:10
- [Mate]: 10-32x1750_shcs_HX-SHCS 0.19-32x1.375x1-C:11 ↔ 10-32 Nylock Nut:12
- [Mate]: 10-32x1750_shcs_HX-SHCS 0.19-32x1.375x1-C:10 ↔ 10-32 Nylock Nut:11
- [Mate]: 1100x215 alum spacer 83062 K-S:11 ↔ 10-32x1750_shcs_HX-SHCS 0.19-32x1.375x1-C:11
- [Mate]: 10-32x1750_shcs_HX-SHCS 0.19-32x1.375x1-C:11 ↔ Bearing Plate:3
- [Mate]: 10-32x1750_shcs_HX-SHCS 0.19-32x1.375x1-C:11 ↔ Bearing Plate:3
- [Mate]: 1100x215 alum spacer 83062 K-S:10 ↔ 10-32x1750_shcs_HX-SHCS 0.19-32x1.375x1-C:12
- [Mate]: 10-32x1750_shcs_HX-SHCS 0.19-32x1.375x1-C:12 ↔ Bearing Plate:3
- [Mate]: 1100x215 alum spacer 83062 K-S:10 ↔ Bearing Plate:3
- [Mate]: 10-32x1750_shcs_HX-SHCS 0.19-32x1.375x1-C:12 ↔ Bearing Plate:3
- [Mate]: 10-32 Nylock Nut:10 ↔ Motor Mount Plate Rev 2:3
- [Mate]: 1100x215 alum spacer 83062 K-S:11 ↔ Bearing Plate:3
- [Mate]: 10-32 Nylock Nut:12 ↔ Motor Mount Plate Rev 2:3
- [Mate]: 10-32x1750_shcs_HX-SHCS 0.19-32x1.375x1-C:9 ↔ Bearing Plate:3
- [Mate]: 10-32 Nylock Nut:9 ↔ 10-32x1750_shcs_HX-SHCS 0.19-32x1.375x1-C:9
- [Mate]: 10-32 Nylock Nut:9 ↔ Motor Mount Plate Rev 2:3
- [Mate]: 10-32x1750_shcs_HX-SHCS 0.19-32x1.375x1-C:9 ↔ Bearing Plate:3
- [Mate]: 1100x215 alum spacer 83062 K-S:9 ↔ 10-32x1750_shcs_HX-SHCS 0.19-32x1.375x1-C:9
- [Mate]: 1100x215 alum spacer 83062 K-S:9 ↔ Bearing Plate:3
- [Mate]: 10-32x1750_shcs_HX-SHCS 0.19-32x1.375x1-C:10 ↔ Bearing Plate:3
- [Mate]: 10-32x1750_shcs_HX-SHCS 0.19-32x1.375x1-C:10 ↔ Bearing Plate:3
- [Mate]: 1100x215 alum spacer 83062 K-S:12 ↔ 10-32x1750_shcs_HX-SHCS 0.19-32x1.375x1-C:10
- [Mate]: 1100x215 alum spacer 83062 K-S:12 ↔ Bearing Plate:3
- [Mate]: 10-32 Nylock Nut:11 ↔ Motor Mount Plate Rev 2:3
- [Mate]: CIM Motor SW:3 ↔ 10-32x0625_shcs_HX-SHCS 0.19-32x1.375x1-C:18
- [Mate]: Motor Mount Plate Rev 2:3 ↔ 10-32x0625_shcs_HX-SHCS 0.19-32x1.375x1-C:18
- [Mate]: Motor Mount Plate Rev 2:3 ↔ 10-32x0625_shcs_HX-SHCS 0.19-32x1.375x1-C:18
- [Mate]: CIM Motor SW:3 ↔ 10-32x0625_shcs_HX-SHCS 0.19-32x1.375x1-C:17
- [Mate]: Motor Mount Plate Rev 2:3 ↔ 10-32x0625_shcs_HX-SHCS 0.19-32x1.375x1-C:17
- [Mate]: Motor Mount Plate Rev 2:3 ↔ 10-32x0625_shcs_HX-SHCS 0.19-32x1.375x1-C:17
- [Mate]: 12T CIM Shaft:3 ↔ CIM Motor SW:3
- [Mate]: VEX 217-2736 0500 Collar Clamp:3 ↔ CIM Motor SW:3
- [Mate]: VEX 217-2736 0500 Collar Clamp:3 ↔ Motor Mount Plate Rev 2:3
- [Mate]: 12T CIM Shaft:3 ↔ CIM Motor SW:3
- [Mate]: CIM Motor SW:3 ↔ Motor Mount Plate Rev 2:3
- [Mate]: PG-71:3 ↔ 375 External Self Locking Ring_98430A134:3
- [Mate]: 48T 10mm bore gear:3 ↔ PG-71:3
- [Mate]: 10-32x1750_shcs_HX-SHCS 0.19-32x1.375x1-C:9 ↔ Motor Mount Plate Rev 2:3
- [Mate]: 10-32x1750_shcs_HX-SHCS 0.19-32x1.375x1-C:12 ↔ Motor Mount Plate Rev 2:3
- [Mate]: 1100x215 alum spacer 83062 K-S:9 ↔ Motor Mount Plate Rev 2:3
- [Mate]: PG-71:3 ↔ 438x406 spacer 13RS100043:3
- [Mate]: Motor Mount Plate Rev 2:3 ↔ 438x406 spacer 13RS100043:3
- [Mate]: Motor Mount Plate Rev 2:3 ↔ SHCS M4x10_91290A187:10
- [Mate]: Motor Mount Plate Rev 2:3 ↔ SHCS M4x10_91290A187:9
- [Mate]: Motor Mount Plate Rev 2:3 ↔ SHCS M4x10_91290A187:12
- [Mate]: Motor Mount Plate Rev 2:3 ↔ SHCS M4x10_91290A187:11
- [Mate]: Motor Mount Plate Rev 2:3 ↔ SHCS M4x10_91290A187:9
- [Mate]: Motor Mount Plate Rev 2:3 ↔ SHCS M4x10_91290A187:10
- [Mate]: Motor Mount Plate Rev 2:3 ↔ SHCS M4x10_91290A187:12
- [Mate]: Motor Mount Plate Rev 2:3 ↔ SHCS M4x10_91290A187:11
- [Mate]: PG-71:3 ↔ 438x406 spacer 13RS100043:3
- [Mate]: Motor Mount Plate Rev 2:3 ↔ PG-71:3
- [Mate]: 48T 10mm bore gear:3 ↔ 438x406 spacer 13RS100043:3
- [Mate]: PG-71:3 ↔ 375 External Self Locking Ring_98430A134:3
- [RelateRotation] (1 ul): 20t 1-25mod bevel gear:3 ↔ 40t 1-25mod bevel gear:3
- [Mate]: 20t 1-25mod bevel gear:3 ↔ Bevel Input Shaft:3
- [RelateRotation] (1 ul): 40T Sleeve Gear REV2:3 ↔ 48T 10mm bore gear:3
- [Mate]: 48T 10mm bore gear:3 ↔ PG-71:3
- [Mate]: 10-24 Hex Washer Rolling x 3-4_93882A213:18 ↔ 4 in HiGrip Wheel:3
- [Mate]: 10-24 Hex Washer Rolling x 3-4_93882A213:17 ↔ 4 in HiGrip Wheel:3
- [Mate]: 10-24 Hex Washer Rolling x 3-4_93882A213:16 ↔ 4 in HiGrip Wheel:3
- [Mate]: 375 Hex Hub:3 ↔ 4 in HiGrip Wheel:3
- [Mate]: 40t 1-25mod bevel gear:3 ↔ 4 in HiGrip Wheel:3
- [Mate]: 375 Hex Hub:4 ↔ 10-24 Hex Washer Rolling x 3-4_93882A213:24
- [Mate]: 375 Hex Hub:4 ↔ 10-24 Hex Washer Rolling x 3-4_93882A213:19
- [Mate]: 375 Hex Hub:4 ↔ 10-24 Hex Washer Rolling x 3-4_93882A213:23
- [Mate]: 375 Hex Hub:4 ↔ 10-24 Hex Washer Rolling x 3-4_93882A213:22
- [Mate]: 375 Hex Hub:4 ↔ 10-24 Hex Washer Rolling x 3-4_93882A213:21
- [Mate]: 375 Hex Hub:4 ↔ 10-24 Hex Washer Rolling x 3-4_93882A213:20
- [Mate]: 375 Hex Hub:4 ↔ 10-24 Hex Washer Rolling x 3-4_93882A213:20
- [Mate]: 375 Hex Hub:4 ↔ 10-24 Hex Washer Rolling x 3-4_93882A213:22
- [Mate]: 375 Hex Hub:4 ↔ 10-24 Hex Washer Rolling x 3-4_93882A213:21
- [Mate]: 375 Hex Hub:4 ↔ 10-24 Hex Washer Rolling x 3-4_93882A213:19
- [Mate]: 375 Hex Hub:4 ↔ 10-24 Hex Washer Rolling x 3-4_93882A213:24
- [Mate]: 375 Hex Hub:4 ↔ 10-24 Hex Washer Rolling x 3-4_93882A213:23
- [Mate]: 375 Hex Output Shaft Rev 2:4 ↔ 375 Hex Hub:4
- [Mate]: 375 Hex Output Shaft Rev 2:4 ↔ 375 Hex Hub:4
- [Mate]: FR6ZZ-L Hex Bearing:7 ↔ 375 Hex Output Shaft Rev 2:4
- [Mate]: FR6ZZ-L Hex Bearing:7 ↔ 375 Hex Output Shaft Rev 2:4
- [Mate]: 375 Hex Output Shaft Rev 2:4 ↔ 40t 1-25mod bevel gear:4
- [Mate]: 375 Hex Output Shaft Rev 2:4 ↔ 40t 1-25mod bevel gear:4
- [RevoluteJoint]: FR6ZZ-L Hex Bearing:8 ↔ AMS C Housing Rev 2:4
- [RevoluteJoint]: FR6ZZ-L Hex Bearing:7 ↔ AMS C Housing Rev 2:4
- [Mate]: FR6ZZ-L Hex Bearing:7 ↔ 125x443 spacer SPS-0750-0443-0125:4
- [Mate]: FR6ZZ-L Hex Bearing:7 ↔ 125x443 spacer SPS-0750-0443-0125:4
- [Mate]: 375 Hex Output Shaft Rev 2:4 ↔ 375 E-klip - Mcm 97431A320_97431A320:4
- [Mate]: 375 Hex Output Shaft Rev 2:4 ↔ 375 E-klip - Mcm 97431A320_97431A320:4
- [Mate]: 375 Hex Hub:4 ↔ 125x443 spacer SPS-0750-0443-0125:4
- [Flush]: FR6ZZ-L Hex Bearing:7 ↔ 375 Hex Output Shaft Rev 2:4
- [RevoluteJoint]: 10-32 Nylock Nut 1_90631A411:13 ↔ 10-32x1250_shcs:15
- [RevoluteJoint]: 10-32 Nylock Nut 1_90631A411:14 ↔ 10-32x1250_shcs:16
- [RevoluteJoint]: 10-32 Nylock Nut 1_90631A411:16 ↔ 10-32x1250_shcs:14
- [RevoluteJoint]: 10-32 Nylock Nut 1_90631A411:15 ↔ 10-32x1250_shcs:13
- [Mate]: 10-32x1250_shcs:14 ↔ Gear Plate:4
- [Mate]: 10-32x1250_shcs:14 ↔ 620x215 alum spacer 83062 K-S:14
- [Flush]: 10-32x1250_shcs:14 ↔ Gear Plate:4
- [Mate]: 620x215 alum spacer 83062 K-S:14 ↔ Gear Plate:4
- [Mate]: 10-32x1250_shcs:13 ↔ Gear Plate:4
- [Mate]: 10-32x1250_shcs:13 ↔ 620x215 alum spacer 83062 K-S:13
- [Flush]: 10-32x1250_shcs:13 ↔ Gear Plate:4
- [Mate]: 620x215 alum spacer 83062 K-S:13 ↔ Gear Plate:4
- [Mate]: 10-32x1250_shcs:15 ↔ Gear Plate:4
- [Flush]: 10-32x1250_shcs:15 ↔ Gear Plate:4
- [Mate]: 10-32x1250_shcs:15 ↔ 620x215 alum spacer 83062 K-S:15
- [Mate]: 620x215 alum spacer 83062 K-S:15 ↔ Gear Plate:4
- [Mate]: 10-32x1250_shcs:16 ↔ 620x215 alum spacer 83062 K-S:16
- [Flush]: 10-32x1250_shcs:16 ↔ Gear Plate:4
- [Mate]: 10-32x1250_shcs:16 ↔ Gear Plate:4
- [Mate]: 620x215 alum spacer 83062 K-S:16 ↔ Gear Plate:4
- [Mate]: FR8ZZ Bearing_smart:4 ↔ 12T CIM Shaft:4
- [Mate]: FR8ZZ Bearing_smart:4 ↔ 12T CIM Shaft:4
- [Mate]: 12T CIM Shaft:4 ↔ Gear Plate:4
- [Mate]: Bevel Input Shaft:4 ↔ FR6ZZ Bearing_smart:7
- [Mate]: Bevel Input Shaft:4 ↔ 500 Washer am-1001:7
- [Mate]: Bevel Input Shaft:4 ↔ 40T 20dp 375h_Inch - Spur gear 20DP 40T 14.5PA .372FW ---S40N3.0H2.0L0.25N:4
- [Mate]: Bevel Input Shaft:4 ↔ 40T 20dp 375h_Inch - Spur gear 20DP 40T 14.5PA .372FW ---S40N3.0H2.0L0.25N:4
- [Flush]: Bevel Input Shaft:4 ↔ 40T 20dp 375h_Inch - Spur gear 20DP 40T 14.5PA .372FW ---S40N3.0H2.0L0.25N:4
- [Mate]: Bevel Input Shaft:4 ↔ 500 Washer am-1001:8
- [Mate]: Bevel Input Shaft:4 ↔ FR6ZZ Bearing_smart:8
- [Mate]: 500 Washer am-1001:8 ↔ FR6ZZ Bearing_smart:8
- [Mate]: Bevel Input Shaft:4 ↔ 500 Washer am-1001:8
- [Flush]: Bevel Input Shaft:4 ↔ 500 Washer am-1001:7
- [Mate]: Gear Plate:4 ↔ FR6ZZ Bearing_smart:8
- [Mate]: Gear Plate:4 ↔ FR6ZZ Bearing_smart:8
- [RevoluteJoint]: 20t 1-25mod bevel gear:4 ↔ Bevel Input Shaft:4
- [Mate]: Gear Plate:4 ↔ 10-32x0625_shcs_HX-SHCS 0.19-32x1.375x1-C:21
- [Flush]: Gear Plate:4 ↔ 10-32x0625_shcs_HX-SHCS 0.19-32x1.375x1-C:21
- [Mate]: Gear Plate:4 ↔ 10-32x0625_shcs_HX-SHCS 0.19-32x1.375x1-C:20
- [Flush]: Gear Plate:4 ↔ 10-32x0625_shcs_HX-SHCS 0.19-32x1.375x1-C:20
- [Mate]: Gear Plate:4 ↔ 10-32x0625_shcs_HX-SHCS 0.19-32x1.375x1-C:19
- [Flush]: Gear Plate:4 ↔ 10-32x0625_shcs_HX-SHCS 0.19-32x1.375x1-C:19
- [Mate]: Gear Plate:4 ↔ 10-32x0625_shcs_HX-SHCS 0.19-32x1.375x1-C:22
- [Flush]: Gear Plate:4 ↔ 10-32x0625_shcs_HX-SHCS 0.19-32x1.375x1-C:22
- [Mate]: FR6ZZ Bearing_smart:7 ↔ 500 Washer am-1001:7
- [Mate]: AMS C Housing Rev 2:4 ↔ 10-32x1250_shcs:14
- [Mate]: AMS C Housing Rev 2:4 ↔ 10-32x1250_shcs:13
- [Mate]: AMS C Housing Rev 2:4 ↔ FR6ZZ Bearing_smart:7
- [Mate]: AMS C Housing Rev 2:4 ↔ FR8ZZ Bearing_smart:4
- [Mate]: 10-32x0625_shcs_HX-SHCS 0.19-32x1.375x1-C:21 ↔ 40T Sleeve Gear REV2:4
- [Mate]: 10-32x0625_shcs_HX-SHCS 0.19-32x1.375x1-C:22 ↔ 40T Sleeve Gear REV2:4
- [Mate]: 10-32x0625_shcs_HX-SHCS 0.19-32x1.375x1-C:19 ↔ 40T Sleeve Gear REV2:4
- [Mate]: 10-32x0625_shcs_HX-SHCS 0.19-32x1.375x1-C:20 ↔ 40T Sleeve Gear REV2:4
- [Mate]: 12T CIM Shaft:4 ↔ 40T Sleeve Gear REV2:4
- [Mate]: Gear Plate:4 ↔ 40T Sleeve Gear REV2:4
- [Mate]: 10-32 Nylock Nut:13 ↔ 10-32x1750_shcs_HX-SHCS 0.19-32x1.375x1-C:13
- [Mate]: 10-32x1750_shcs_HX-SHCS 0.19-32x1.375x1-C:16 ↔ 10-32 Nylock Nut:14
- [Mate]: 10-32x1750_shcs_HX-SHCS 0.19-32x1.375x1-C:15 ↔ 10-32 Nylock Nut:16
- [Mate]: 10-32x1750_shcs_HX-SHCS 0.19-32x1.375x1-C:14 ↔ 10-32 Nylock Nut:15
- [Mate]: 1100x215 alum spacer 83062 K-S:15 ↔ 10-32x1750_shcs_HX-SHCS 0.19-32x1.375x1-C:15
- [Mate]: 10-32x1750_shcs_HX-SHCS 0.19-32x1.375x1-C:15 ↔ Bearing Plate:4
- [Mate]: 10-32x1750_shcs_HX-SHCS 0.19-32x1.375x1-C:15 ↔ Bearing Plate:4
- [Mate]: 1100x215 alum spacer 83062 K-S:14 ↔ 10-32x1750_shcs_HX-SHCS 0.19-32x1.375x1-C:16
- [Mate]: 10-32x1750_shcs_HX-SHCS 0.19-32x1.375x1-C:16 ↔ Bearing Plate:4
- [Mate]: 1100x215 alum spacer 83062 K-S:14 ↔ Bearing Plate:4
- [Mate]: 10-32x1750_shcs_HX-SHCS 0.19-32x1.375x1-C:16 ↔ Bearing Plate:4